# Autodesk Inventor assembly: FrameV3
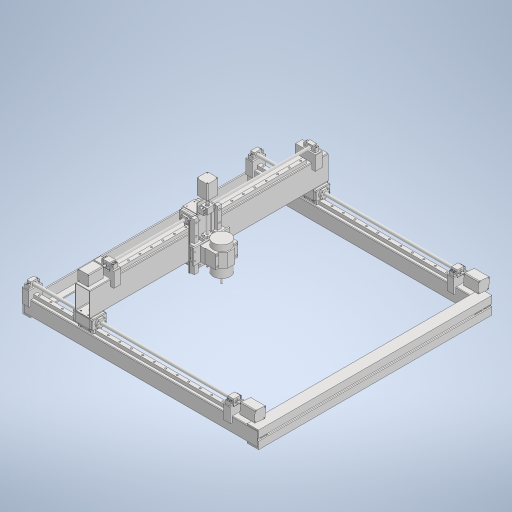
[picture p0: Inventor's stored thumbnail of the model, 512x512]
Saved by Autodesk Inventor 2023 (Build 270158000, 158)
## iProperties
Created: 2022-05-03
Part Number: FrameV3
Document SubType Name: Assembly
Designer: plebbb
Author: plebbb
## Documents named in this file (31)
- D:\Users\plebbb\Desktop\CNC_Project\FrameV3.iam
- D:\Users\plebbb\Desktop\CNC_Project\Ballscrew_Assembly.iam
- D:\Users\plebbb\Desktop\CNC_Project\X_GANTRY.iam
- D:\Users\plebbb\Desktop\CNC_Project\Steel_L_Bracket.ipt
- D:\Users\plebbb\Desktop\CNC_Project\5x3_Tube.ipt
- D:\Users\plebbb\Desktop\CNC_Project\HGW20CC_Rail_800mm.ipt
- D:\Users\plebbb\Desktop\CNC_Project\BF10.ipt
- D:\Users\plebbb\Desktop\CNC_Project\BK10.ipt
- D:\Users\plebbb\Desktop\CNC_Project\SFU1204-500.ipt
- D:\Users\plebbb\Desktop\CNC_Project\Ballscrew_Assembly_1204.iam
- D:\Users\plebbb\Desktop\CNC_Project\HGW20CC_Slider.ipt
- D:\Users\plebbb\Desktop\CNC_Project\Flat_Plate.ipt
- D:\Users\plebbb\Desktop\CNC_Project\L_Bracketr.ipt
- D:\Users\plebbb\Desktop\CNC_Project\HGW20CC_Rail_300mm.ipt
- D:\Users\plebbb\Desktop\CNC_Project\Spindle.ipt
- D:\Users\plebbb\Desktop\CNC_Project\Spindle_Holder.ipt
- D:\Users\plebbb\Desktop\CNC_Project\BF10_Spacer.ipt
- D:\Users\plebbb\Desktop\CNC_Project\BK10_Spacer.ipt
- D:\Users\plebbb\Desktop\CNC_Project\Rail_Spacer_Plate.ipt
- D:\Users\plebbb\Desktop\CNC_Project\Spindle_Mounting_Plate.ipt
- D:\Users\plebbb\Desktop\CNC_Project\DSG12H.ipt
- D:\Users\plebbb\Desktop\CNC_Project\SFU1204_Nut.ipt
- D:\Users\plebbb\Desktop\CNC_Project\Nema23.ipt
- D:\Users\plebbb\Desktop\CNC_Project\SFU1204-300.ipt
- D:\Users\plebbb\Desktop\CNC_Project\Z_Screw_Holder_Bracket.ipt
- D:\Users\plebbb\Desktop\CNC_Project\FrameV3\AIP\FEA\dyol7vh0g.fins
- D:\Users\plebbb\Desktop\CNC_Project\FrameV3\AIP\FEA\dyol7vh0g.fsat
- D:\Users\plebbb\Desktop\CNC_Project\FrameV3\AIP\FEA\dyol7vh0g.ftes
- D:\Users\plebbb\Desktop\CNC_Project\FrameV3\AIP\FEA\dyol7vh0g.fwiz
- D:\Users\plebbb\Desktop\CNC_Project\FrameV3\AIP\FEA\dyol7vheo.fmsh
- D:\Users\plebbb\Desktop\CNC_Project\FrameV3\AIP\FEA\dyol7vhep.fres
## Components (35 placed, 24 different names)
1. Ballscrew_Assembly:1 [sub-assembly] — Flush:11, Mate:66, Mate:67
2. X_GANTRY:1 [sub-assembly] — Mate:30, Mate:31, Flush:4, Mate:32, Mate:33, Flush:5, Mate:38, Flush:9, Mate:40, Flush:49
3. X_GANTRY:2 [sub-assembly] — Mate:25, Mate:26, Mate:27, Mate:28, Mate:29, Mate:34, Mate:35, Mate:36, Mate:37, Flush:6, Flush:7, Mate:39, Flush:8
4. Ballscrew_Assembly:2 [sub-assembly] — Mate:25, Mate:26, Mate:27, Mate:28, Mate:29, Mate:43, Mate:68
5. Steel_L_Bracket:1 — Mate:30, Mate:31, Flush:4, Mate:34, Mate:37, Flush:6, Flush:42, Mate:42, Mate:69
6. Steel_L_Bracket:2 — Mate:32, Mate:33, Flush:5, Mate:35, Mate:36, Flush:7
7. Steel_L_Bracket:3 — Mate:38, Mate:39, Flush:8, Flush:9, Mate:40
8. 5x3_Tube:1 — Mate:43, Flush:11, Mate:47, Mate:55, Flush:13, Flush:14, Mate:66, Mate:67, Mate:68, Mate:74, Mate:78, Mate:79, Flush:44
9. HGW20CC_Rail_800mm:1 — Mate:55, Mate:56, Mate:57, Flush:12, Flush:14, Flush:53
10. HGW20CC_Rail_800mm:2 — Mate:47, Mate:48, Mate:49, Flush:12, Flush:13, Flush:53, Mate:104
11. BF10:1 — Mate:53, Mate:54, Mate:75, Mate:76, Mate:77
12. BK10:1 — Mate:51, Mate:52, Mate:71, Mate:72, Mate:73, Mate:88
13. SFU1204-500:1 — Mate:50, Mate:51, Mate:52, Mate:53, Mate:54, Mate:105, Mate:106
14. Ballscrew_Assembly_1204:1 [sub-assembly] — Mate:48, Mate:49, Mate:50, Mate:58, Flush:15, Mate:88, Mate:89, Mate:102, Mate:103, Mate:112, Mate:113, Mate:114
15. HGW20CC_Slider:1 — Mate:56, Mate:57, Mate:60, Mate:61, Mate:62
16. Flat_Plate:1 — Mate:58, Mate:63, Flush:15, Angle:2, Flush:45, Mate:80, Mate:81, Flush:46, Flush:47, Flush:48, Mate:82, Mate:83, Angle:3, Flush:50, Flush:51, Mate:102, Mate:103, Mate:107, Mate:108, Flush:54
17. L_Bracketr:1 — Mate:60, Mate:61, Mate:62, Mate:63, Mate:82, Mate:83
18. HGW20CC_Rail_300mm:1 — Mate:64, Angle:1, Angle:2, Flush:16, Mate:84, Mate:85, Flush:50, Flush:51
19. HGW20CC_Rail_300mm:2 — Mate:65, Angle:1, Flush:16, Mate:86, Mate:87, Flush:52
20. Spindle:1 — Mate:70, Flush:43, Flush:49
21. Spindle_Holder:1 — Mate:70, Flush:43, Angle:3, Mate:90, Mate:91, Mate:92
22. BF10_Spacer:1 — Mate:75, Mate:76, Mate:77, Mate:78, Mate:79, Flush:44, Mate:89, Mate:107
23. BK10_Spacer:1 — Mate:71, Mate:72, Mate:73, Mate:74, Mate:104, Mate:108
24. Rail_Spacer_Plate:1 — Mate:81, Flush:46, Flush:48, Mate:65
25. Rail_Spacer_Plate:2 — Flush:45, Mate:80, Flush:47, Mate:64
26. HGW20CC_Slider:2 — Mate:84, Mate:85, Mate:94, Mate:95
27. HGW20CC_Slider:3 — Mate:86, Mate:87, Mate:93, Flush:52
28. Spindle_Mounting_Plate:1 — Mate:90, Mate:91, Mate:92, Mate:93, Mate:94, Mate:95, Mate:96, Mate:97, Mate:98
29. DSG12H:1 — Mate:96, Mate:97, Mate:98, Mate:99, Mate:100, Mate:101
30. SFU1204_Nut:1 — Mate:99, Mate:100, Mate:101, Mate:109, Mate:118
31. Nema23:1 — Mate:105, Mate:106
32. SFU1204-300:1 — Mate:109, Flush:54, Mate:110, Mate:111, Mate:116, Mate:117
33. Nema23:2 — Mate:116, Mate:117
34. BK10:2 — Mate:110, Mate:111, Mate:115, Mate:118
35. Z_Screw_Holder_Bracket:1 — Mate:112, Mate:113, Mate:114, Mate:115
## Relationships (125: Mate 95, Flush 27, Angle 3)
- [Mate]: Ballscrew_Assembly:1 ↔ X_GANTRY:1
- [Mate]: Ballscrew_Assembly:1 ↔ X_GANTRY:1
- [Flush]: Ballscrew_Assembly:1 ↔ X_GANTRY:1
- [Flush]: Ballscrew_Assembly:1 ↔ X_GANTRY:1
- [Mate]: Ballscrew_Assembly:1 ↔ X_GANTRY:1
- [Mate]: Ballscrew_Assembly:1 ↔ X_GANTRY:1
- [Mate]: Ballscrew_Assembly:1 ↔ X_GANTRY:1
- [Mate]: Ballscrew_Assembly:1 ↔ X_GANTRY:1
- Mate:25: X_GANTRY:2 ↔ Ballscrew_Assembly:2
- Mate:26: X_GANTRY:2 ↔ Ballscrew_Assembly:2
- Mate:27: X_GANTRY:2 ↔ Ballscrew_Assembly:2
- Mate:28: X_GANTRY:2 ↔ Ballscrew_Assembly:2
- Mate:29: X_GANTRY:2 ↔ Ballscrew_Assembly:2
- Mate:30: X_GANTRY:1 ↔ Steel_L_Bracket:1
- Mate:31: X_GANTRY:1 ↔ Steel_L_Bracket:1
- Flush:4: X_GANTRY:1 ↔ Steel_L_Bracket:1
- Mate:32: X_GANTRY:1 ↔ Steel_L_Bracket:2
- Mate:33: X_GANTRY:1 ↔ Steel_L_Bracket:2
- Flush:5: X_GANTRY:1 ↔ Steel_L_Bracket:2
- Mate:34: X_GANTRY:2 ↔ Steel_L_Bracket:1
- Mate:35: X_GANTRY:2 ↔ Steel_L_Bracket:2
- Mate:36: X_GANTRY:2 ↔ Steel_L_Bracket:2
- Mate:37: X_GANTRY:2 ↔ Steel_L_Bracket:1
- Flush:6: X_GANTRY:2 ↔ Steel_L_Bracket:1
- Flush:7: X_GANTRY:2 ↔ Steel_L_Bracket:2
- Mate:38: X_GANTRY:1 ↔ Steel_L_Bracket:3
- Mate:39: X_GANTRY:2 ↔ Steel_L_Bracket:3
- Flush:8: X_GANTRY:2 ↔ Steel_L_Bracket:3
- Flush:9: X_GANTRY:1 ↔ Steel_L_Bracket:3
- Mate:40: X_GANTRY:1 ↔ Steel_L_Bracket:3
- Flush:42: Steel_L_Bracket:1
- Mate:42: Steel_L_Bracket:1
- Mate:69: Steel_L_Bracket:1
- Mate:43: Ballscrew_Assembly:2 ↔ 5x3_Tube:1
- Flush:11: Ballscrew_Assembly:1 ↔ 5x3_Tube:1
- Mate:47: 5x3_Tube:1 ↔ HGW20CC_Rail_800mm:2
- Mate:48: HGW20CC_Rail_800mm:2 ↔ Ballscrew_Assembly_1204:1
- Mate:49: HGW20CC_Rail_800mm:2 ↔ Ballscrew_Assembly_1204:1
- Mate:50: SFU1204-500:1 ↔ Ballscrew_Assembly_1204:1
- Mate:51: BK10:1 ↔ SFU1204-500:1
- Mate:52: BK10:1 ↔ SFU1204-500:1
- Mate:53: BF10:1 ↔ SFU1204-500:1
- Mate:54: BF10:1 ↔ SFU1204-500:1
- Mate:55: 5x3_Tube:1 ↔ HGW20CC_Rail_800mm:1
- Mate:56: HGW20CC_Rail_800mm:1 ↔ HGW20CC_Slider:1
- Mate:57: HGW20CC_Rail_800mm:1 ↔ HGW20CC_Slider:1
- Flush:12: HGW20CC_Rail_800mm:1 ↔ HGW20CC_Rail_800mm:2
- Flush:13 (-10 mm): 5x3_Tube:1 ↔ HGW20CC_Rail_800mm:2
- Flush:14 (28.1 mm): 5x3_Tube:1 ↔ HGW20CC_Rail_800mm:1
- Mate:58: Ballscrew_Assembly_1204:1 ↔ Flat_Plate:1
- Mate:60: HGW20CC_Slider:1 ↔ L_Bracketr:1
- Mate:61: HGW20CC_Slider:1 ↔ L_Bracketr:1
- Mate:62: HGW20CC_Slider:1 ↔ L_Bracketr:1
- Mate:63: Flat_Plate:1 ↔ L_Bracketr:1
- Flush:15: Ballscrew_Assembly_1204:1 ↔ Flat_Plate:1
- Mate:64: HGW20CC_Rail_300mm:1 ↔ Rail_Spacer_Plate:2
- Mate:65: HGW20CC_Rail_300mm:2 ↔ Rail_Spacer_Plate:1
- Angle:1 (0 deg): HGW20CC_Rail_300mm:1 ↔ HGW20CC_Rail_300mm:2
- Angle:2 (0 deg): Flat_Plate:1 ↔ HGW20CC_Rail_300mm:1
- Flush:16: HGW20CC_Rail_300mm:1 ↔ HGW20CC_Rail_300mm:2
- Mate:66: Ballscrew_Assembly:1 ↔ 5x3_Tube:1
- Mate:67: Ballscrew_Assembly:1 ↔ 5x3_Tube:1
- Mate:68: Ballscrew_Assembly:2 ↔ 5x3_Tube:1
- Mate:70: Spindle:1 ↔ Spindle_Holder:1
- Flush:43 (50 mm): Spindle:1 ↔ Spindle_Holder:1
- Mate:71: BK10:1 ↔ BK10_Spacer:1
- Mate:72: BK10:1 ↔ BK10_Spacer:1
- Mate:73: BK10:1 ↔ BK10_Spacer:1
- Mate:74: 5x3_Tube:1 ↔ BK10_Spacer:1
- Mate:75: BF10:1 ↔ BF10_Spacer:1
- Mate:76: BF10:1 ↔ BF10_Spacer:1
- Mate:77: BF10:1 ↔ BF10_Spacer:1
- Mate:78: 5x3_Tube:1 ↔ BF10_Spacer:1
- Mate:79: 5x3_Tube:1 ↔ BF10_Spacer:1
- Flush:44 (50 mm): 5x3_Tube:1 ↔ BF10_Spacer:1
- Flush:45: Flat_Plate:1 ↔ Rail_Spacer_Plate:2
- Mate:80: Flat_Plate:1 ↔ Rail_Spacer_Plate:2
- Mate:81: Flat_Plate:1 ↔ Rail_Spacer_Plate:1
- Flush:46: Flat_Plate:1 ↔ Rail_Spacer_Plate:1
- Flush:47: Flat_Plate:1 ↔ Rail_Spacer_Plate:2
- Flush:48: Flat_Plate:1 ↔ Rail_Spacer_Plate:1
- Mate:82: Flat_Plate:1 ↔ L_Bracketr:1
- Mate:83: Flat_Plate:1 ↔ L_Bracketr:1
- Mate:84: HGW20CC_Rail_300mm:1 ↔ HGW20CC_Slider:2
- Mate:85: HGW20CC_Rail_300mm:1 ↔ HGW20CC_Slider:2
- Mate:86: HGW20CC_Rail_300mm:2 ↔ HGW20CC_Slider:3
- Mate:87: HGW20CC_Rail_300mm:2 ↔ HGW20CC_Slider:3
- Angle:3 (0 deg): Flat_Plate:1 ↔ Spindle_Holder:1
- Mate:88: BK10:1 ↔ Ballscrew_Assembly_1204:1
- Mate:89: Ballscrew_Assembly_1204:1 ↔ BF10_Spacer:1
- Mate:90: Spindle_Holder:1 ↔ Spindle_Mounting_Plate:1
- Mate:91: Spindle_Holder:1 ↔ Spindle_Mounting_Plate:1
- Mate:92: Spindle_Holder:1 ↔ Spindle_Mounting_Plate:1
- Mate:93: HGW20CC_Slider:3 ↔ Spindle_Mounting_Plate:1
- Mate:94: HGW20CC_Slider:2 ↔ Spindle_Mounting_Plate:1
- Mate:95: HGW20CC_Slider:2 ↔ Spindle_Mounting_Plate:1
- Flush:49: X_GANTRY:1 ↔ Spindle:1
- Mate:96: Spindle_Mounting_Plate:1 ↔ DSG12H:1
- Mate:97: Spindle_Mounting_Plate:1 ↔ DSG12H:1
- Mate:98: Spindle_Mounting_Plate:1 ↔ DSG12H:1
- Mate:99: DSG12H:1 ↔ SFU1204_Nut:1
- Mate:100: DSG12H:1 ↔ SFU1204_Nut:1
- Mate:101: DSG12H:1 ↔ SFU1204_Nut:1
- Flush:50: Flat_Plate:1 ↔ HGW20CC_Rail_300mm:1
- Flush:51 (-5.2 mm): Flat_Plate:1 ↔ HGW20CC_Rail_300mm:1
- Mate:102: Ballscrew_Assembly_1204:1 ↔ Flat_Plate:1
- Mate:103: Ballscrew_Assembly_1204:1 ↔ Flat_Plate:1
- Flush:52: HGW20CC_Rail_300mm:2 ↔ HGW20CC_Slider:3
- Flush:53: HGW20CC_Rail_800mm:1 ↔ HGW20CC_Rail_800mm:2
- Mate:104: HGW20CC_Rail_800mm:2 ↔ BK10_Spacer:1
- Mate:105: SFU1204-500:1 ↔ Nema23:1
- Mate:106: SFU1204-500:1 ↔ Nema23:1
- Mate:107: Flat_Plate:1 ↔ BF10_Spacer:1
- Mate:108: Flat_Plate:1 ↔ BK10_Spacer:1
- Mate:109: SFU1204_Nut:1 ↔ SFU1204-300:1
- Flush:54: Flat_Plate:1 ↔ SFU1204-300:1
- Mate:110: SFU1204-300:1 ↔ BK10:2
- Mate:111: SFU1204-300:1 ↔ BK10:2
- Mate:112: Ballscrew_Assembly_1204:1 ↔ Z_Screw_Holder_Bracket:1
- Mate:113: Ballscrew_Assembly_1204:1 ↔ Z_Screw_Holder_Bracket:1
- Mate:114: Ballscrew_Assembly_1204:1 ↔ Z_Screw_Holder_Bracket:1
- Mate:115: BK10:2 ↔ Z_Screw_Holder_Bracket:1
- Mate:116: SFU1204-300:1 ↔ Nema23:2
- Mate:117: SFU1204-300:1 ↔ Nema23:2
- Mate:118: SFU1204_Nut:1 ↔ BK10:2
## Named parameters: sa_0 = 100000
note: some values were not read from the file. Shown as the stored number, unit unknown: "sa_0".
